# Autodesk Inventor assembly: Final-ass
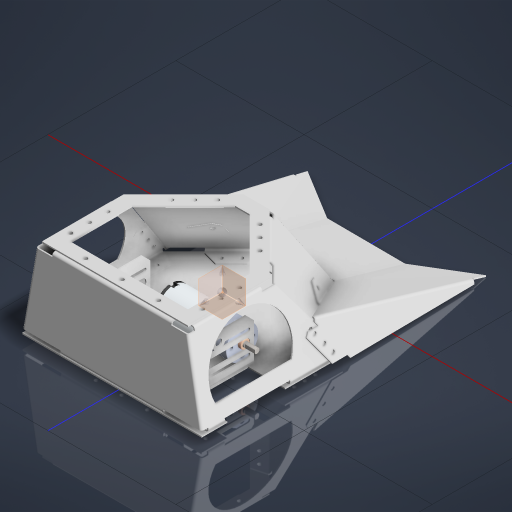
[picture p0: Inventor's stored thumbnail of the model, 512x512]
Saved by Autodesk Inventor 2023 (Build 270158000, 158)
## iProperties
Created: 2022-05-30
Part Number: Final-ass
Document SubType Name: Assembly
Designer: x43dn
Author: x43dn
## Documents named in this file (8)
- C:\Users\x43dn\Desktop\sumoltaneous-equations\sumoltaneous-equations-inventor\Final-ass.iam
- C:\Users\x43dn\Desktop\sumoltaneous-equations\sumoltaneous-equations-inventor\Bottomp.ipt
- C:\Users\x43dn\Desktop\sumoltaneous-equations\sumoltaneous-equations-inventor\Frontp.ipt
- C:\Users\x43dn\Desktop\sumoltaneous-equations\sumoltaneous-equations-inventor\Backp.ipt
- C:\Users\x43dn\Desktop\sumoltaneous-equations\sumoltaneous-equations-inventor\Topp.ipt
- C:\Users\x43dn\Desktop\sumoltaneous-equations\sumoltaneous-equations-inventor\Rampp.ipt
- C:\Users\x43dn\Desktop\sumoltaneous-equations\sumoltaneous-equations-inventor\Motor-mountp.ipt
- C:\Users\x43dn\Desktop\sumoltaneous-equations\sumoltaneous-equations-inventor\JGA25-370.ipt
## Components (8 placed, 7 different names)
1. Bottomp:1 — Mate:1, Mate:2, Mate:3, Mate:4, Mate:8
2. Frontp:1 — Mate:1, Mate:2, Mate:7
3. Backp:1 — Mate:3, Mate:4, Mate:5, Mate:6
4. Topp:1 — Mate:5, Mate:6
5. Rampp:1 — Mate:7
6. Motor-mountp:1 — Mate:8, Insert:1, Insert:2
7. JGA25-370:1 — Insert:1
8. JGA25-370:2 — Insert:2
## Relationships (10: Mate 8, Insert 2)
- Mate:1: Bottomp:1 ↔ Frontp:1
- Mate:2: Bottomp:1 ↔ Frontp:1
- Mate:3: Bottomp:1 ↔ Backp:1
- Mate:4: Bottomp:1 ↔ Backp:1
- Mate:5: Backp:1 ↔ Topp:1
- Mate:6: Backp:1 ↔ Topp:1
- Mate:7: Frontp:1 ↔ Rampp:1
- Mate:8: Bottomp:1 ↔ Motor-mountp:1
- Insert:1: Motor-mountp:1 ↔ JGA25-370:1
- Insert:2: Motor-mountp:1 ↔ JGA25-370:2
